# Autodesk Inventor assembly: WheelAssembly
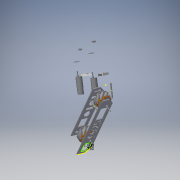
[picture p0: Inventor's stored thumbnail of the model, 180x180]
Saved by Autodesk Inventor 2017 (Build 210142000, 142)
## iProperties
Created: 2016-09-10
Part Number: WheelAssembly
Document SubType Name: Assembly
Designer: RoboticsUser
Author: RoboticsUser
## Documents named in this file (13)
- C:\Robotics\CAD\2016-17_CAD\WheelAssemble2.0 - left - Backup.iam
- C:\Robotics\CAD\COTSParts\Actobotics\545 parts\545556.ipt
- C:\Robotics\CAD\COTSParts\Actobotics\615 parts\615102.ipt
- C:\Robotics\CAD\COTSParts\Actobotics\634 parts\634080.ipt
- C:\Robotics\CAD\COTSParts\Motors\Andymark 2964  NeveRest 40 Motor.ipt
- C:\Robotics\CAD\COTSParts\Tetrix\tetrix-motor-mounts-1.snapshot.1\Tetrex 2pc motor mount.ipt
- C:\Robotics\CAD\COTSParts\Actobotics\545 parts\545456.ipt
- C:\Robotics\CAD\COTSParts\Wheels\AndyMark Mecanum Wheels\100mm Aluminum Mecanum wheels.ipt
- C:\Robotics\CAD\2016-17_CAD\DrainTrainPlate2.0.iam
- C:\Robotics\CAD\2016-17_CAD\DriveTrainPlate -Inside.ipt
- C:\Robotics\CAD\COTSParts\Actobotics\535 parts\535198.ipt
- C:\Robotics\CAD\COTSParts\Actobotics\collar.ipt
- C:\Robotics\CAD\2016-17_CAD\drive train standoff.ipt
## Components (35 placed, 12 different names)
1. 545556:2 — Mate:31, Mate:32, Mate:33, Mate:34, Mate:35
2. 615102:4
3. 634080:2 — Mate:1, Mate:2, Mate:24, Mate:26, Mate:35, Mate:39, Mate:40
4. 545556:6 — Mate:12, Mate:13, Mate:21
5. 634080:3 — Mate:3, Mate:4, Mate:11, Mate:14, Mate:18, Mate:22, Mate:38, Mate:42
6. Andymark 2964  NeveRest 40 Motor:2
7. 545556:8
8. 545556:9
9. Tetrex 2pc motor mount:1
10. Tetrex 2pc motor mount:2
11. 545456:1 — Mate:27, Mate:28, Mate:29
12. 545456:3 — Mate:12, Mate:13, Mate:14, Mate:15
13. 615102:6
14. 615102:7 — Mate:31, Mate:34, Mate:37
15. 100mm Aluminum Mecanum wheels:1 — Mate:11, Mate:15, Mate:19
16. 100mm Aluminum Mecanum wheels:2 — Mate:24, Mate:29, Mate:36
17. 545456:4 — Mate:25, Mate:32, Mate:33, Mate:36
18. 545456:5 — Mate:16, Mate:17, Mate:18, Mate:19
19. 545556:13 — Mate:25, Mate:26, Mate:27, Mate:28, Mate:30
20. 545556:12 — Mate:16, Mate:17, Insert:4
21. DriveTrainPlate -Inside:1 — Mate:2, Mate:4, Mate:9, Mate:10, Mate:37, Insert:5, Insert:6, Mate:43
22. 615102:8 — Mate:38, Insert:4
23. 535198:2 — Insert:6
24. 535198:3 — Insert:5
25. 535198:4 — Insert:3
26. 535198:5 — Insert:2
27. collar:1 — Mate:40, Mate:41
28. collar:2 — Mate:22, Mate:23
29. Andymark 2964  NeveRest 40 Motor:3
30. collar:3 — Mate:9, Mate:39
31. collar:4 — Mate:10, Mate:42
32. drive train standoff:1 — Mate:43
33. drive train standoff:2
34. drive train standoff:3
35. DrainTrainPlate2.0:1 [sub-assembly] — Mate:1, Mate:3, Mate:21, Insert:2, Mate:23, Mate:30, Insert:3, Mate:41
## Relationships (43: Mate 38, Insert 5)
- Mate:1: 634080:2 ↔ DrainTrainPlate2.0:1
- Mate:2: 634080:2 ↔ DriveTrainPlate -Inside:1
- Mate:3: 634080:3 ↔ DrainTrainPlate2.0:1
- Mate:4: 634080:3 ↔ DriveTrainPlate -Inside:1
- Mate:9: DriveTrainPlate -Inside:1 ↔ collar:3
- Mate:10: DriveTrainPlate -Inside:1 ↔ collar:4
- Mate:11: 634080:3 ↔ 100mm Aluminum Mecanum wheels:1
- Mate:12: 545556:6 ↔ 545456:3
- Mate:13: 545556:6 ↔ 545456:3
- Mate:14: 634080:3 ↔ 545456:3
- Mate:15: 545456:3 ↔ 100mm Aluminum Mecanum wheels:1
- Mate:16: 545456:5 ↔ 545556:12
- Mate:17: 545456:5 ↔ 545556:12
- Mate:18: 634080:3 ↔ 545456:5
- Mate:19: 100mm Aluminum Mecanum wheels:1 ↔ 545456:5
- Mate:21 (3.175 mm): 545556:6 ↔ DrainTrainPlate2.0:1
- Insert:2: 535198:5 ↔ DrainTrainPlate2.0:1
- Mate:22: 634080:3 ↔ collar:2
- Mate:23: collar:2 ↔ DrainTrainPlate2.0:1
- Mate:24: 634080:2 ↔ 100mm Aluminum Mecanum wheels:2
- Mate:25: 545456:4 ↔ 545556:13
- Mate:26: 634080:2 ↔ 545556:13
- Mate:27: 545456:1 ↔ 545556:13
- Mate:28: 545456:1 ↔ 545556:13
- Mate:29: 545456:1 ↔ 100mm Aluminum Mecanum wheels:2
- Mate:30 (3.175 mm): 545556:13 ↔ DrainTrainPlate2.0:1
- Mate:31: 545556:2 ↔ 615102:7
- Mate:32: 545556:2 ↔ 545456:4
- Mate:33: 545556:2 ↔ 545456:4
- Mate:34: 545556:2 ↔ 615102:7
- Mate:35: 545556:2 ↔ 634080:2
- Mate:36: 100mm Aluminum Mecanum wheels:2 ↔ 545456:4
- Mate:37 (6.35 mm): 615102:7 ↔ DriveTrainPlate -Inside:1
- Insert:3: 535198:4 ↔ DrainTrainPlate2.0:1
- Mate:38: 634080:3 ↔ 615102:8
- Insert:4: 545556:12 ↔ 615102:8
- Insert:5: DriveTrainPlate -Inside:1 ↔ 535198:3
- Mate:39: 634080:2 ↔ collar:3
- Mate:40: 634080:2 ↔ collar:1
- Mate:41: collar:1 ↔ DrainTrainPlate2.0:1
- Insert:6: DriveTrainPlate -Inside:1 ↔ 535198:2
- Mate:42: 634080:3 ↔ collar:4
- Mate:43: DriveTrainPlate -Inside:1 ↔ drive train standoff:1
